# Autodesk Inventor assembly: Walls
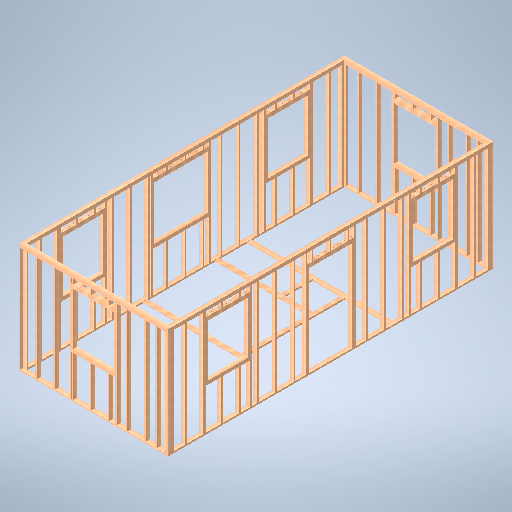
[picture p0: Inventor's stored thumbnail of the model, 512x512]
Saved by Autodesk Inventor 2025.1 (Build 291241020, 241B)
## iProperties
Created: 2024-09-15
Part Number: Walls
Document SubType Name: Assembly
Designer: Tom
Author: Tom
## Documents named in this file (17)
- C:\Users\Tom\Documents\Inventor\Mobility\Additional_Building\Framing_For_First_Floor.iam
- C:\Users\Tom\Documents\Inventor\Mobility\Additional_Building\Plate_With_Length_144_Inches.ipt
- C:\Users\Tom\Documents\Inventor\Mobility\Additional_Building\Plate_With_Length_125_Inches.ipt
- C:\Users\Tom\Documents\Inventor\Mobility\Additional_Building\California_Corner.iam
- C:\Users\Tom\Documents\Inventor\Mobility\Additional_Building\Stud_With_Height_93_Inches.ipt
- C:\Users\Tom\Documents\Inventor\Mobility\Additional_Building\Plate_With_Length_132_Inches.ipt
- C:\Users\Tom\Documents\Inventor\Mobility\Additional_Building\Plate_With_Length_68.5_Inches.ipt
- C:\Users\Tom\Documents\Inventor\Mobility\Additional_Building\Plate_With_Length_86.5625_Inches_And_Image_Of_Bath_Tub.ipt
- C:\Users\Tom\Documents\Inventor\Mobility\Additional_Building\Plate_With_Length_60_Inches.ipt
- C:\Users\Tom\Documents\Inventor\Mobility\Additional_Building\Plate_With_Length_25_Inches.ipt
- C:\Users\Tom\Documents\Inventor\Mobility\Additional_Building\Plate_With_Length_86.5625_Inches.ipt
- C:\Users\Tom\Documents\Inventor\Mobility\Additional_Building\Stud_With_Height_80.5_Inches.ipt
- C:\Users\Tom\Documents\Inventor\Mobility\Additional_Building\Stud_With_Height_9_Inches.ipt
- C:\Users\Tom\Documents\Inventor\Mobility\Additional_Building\Framing_For_First_Floor_Window.iam
- C:\Users\Tom\Documents\Inventor\Mobility\Additional_Building\Framing_For_Side_Window.iam
- C:\Users\Tom\Documents\Inventor\Mobility\Additional_Building\Framing_For_Bathroom_Window.iam
- C:\Users\Tom\Documents\Inventor\Mobility\Additional_Building\Header_With_Dimensions_3.5_x_3.5_x_41.25_Inches.iam
## Components (75 placed, 16 different names)
1. California_Corner:1 [sub-assembly] — Mate:2, Flush:3, Flush:4, Flush:95
2. California_Corner:2 [sub-assembly] — Mate:13, Flush:13, Flush:14, Flush:19, Flush:20, Flush:31, Mate:34, Flush:64, Flush:70
3. California_Corner:3 [sub-assembly] — Mate:14, Flush:15, Flush:16
4. California_Corner:4 [sub-assembly] — Mate:15, Flush:17, Flush:18
5. Plate_With_Length_125_Inches:5 — Mate:16, Flush:22, Mate:17, Mate:19, Mate:24, Flush:27, Flush:45
6. Plate_With_Length_60_Inches:1 — Mate:19, Mate:27, Mate:31, Flush:44
7. Plate_With_Length_25_Inches:1 — Mate:25, Mate:28, Flush:45
8. Plate_With_Length_25_Inches:2 — Mate:24, Flush:27, Mate:25, Mate:29
9. Plate_With_Length_86.5625_Inches_And_Image_Of_Bath_Tub:1 — Mate:26, Flush:28, Mate:27, Mate:28, Mate:29, Flush:44
10. Plate_With_Length_86.5625_Inches:1 — Mate:30, Mate:31, Flush:29, Mate:79
11. Stud_With_Height_93_Inches:56 — Mate:33, Flush:32, Mate:34, Mate:39
12. Stud_With_Height_93_Inches:57 — Mate:36, Flush:35, Mate:41, Mate:80, Flush:87
13. Stud_With_Height_80.5_Inches:1 — Mate:38, Flush:36, Mate:39
14. Stud_With_Height_80.5_Inches:2 — Mate:40, Flush:37, Mate:41, Mate:81
15. Framing_For_Bathroom_Window:1 [sub-assembly] — Mate:78, Flush:86, Mate:79
16. Header_With_Dimensions_3.5_x_3.5_x_41.25_Inches:1 [sub-assembly] — Mate:80, Mate:81, Flush:87
17. Plate_With_Length_132_Inches:1 — Mate:8, Flush:9, Flush:10, Mate:10
18. Plate_With_Length_132_Inches:2
19. Plate_With_Length_144_Inches:9 — Mate:11, Mate:12, Flush:12
20. Plate_With_Length_144_Inches:10
21. Stud_With_Height_9_Inches:1 — Flush:39
22. Stud_With_Height_9_Inches:2
23. Stud_With_Height_9_Inches:3
24. Stud_With_Height_93_Inches:49 — Mate:32, Flush:30, Flush:31
25. Framing_For_Side_Window:1 [sub-assembly] — Mate:65, Flush:69, Flush:70
26. Stud_With_Height_93_Inches:71
27. Framing_For_Side_Window:2 [sub-assembly]
28. Stud_With_Height_93_Inches:1 — Mate:4, Flush:6, Flush:19, Flush:39, Flush:43, Flush:88
29. Stud_With_Height_93_Inches:89 — Mate:84, Flush:93, Mate:85
30. Framing_For_First_Floor_Window:1 [sub-assembly] — Mate:62, Flush:63, Flush:64, Mate:85
31. Framing_For_First_Floor_Window:2 [sub-assembly] — Flush:94, Mate:86, Flush:95, Mate:88, Flush:98
32. Stud_With_Height_93_Inches:90 — Mate:87, Flush:96, Mate:88
33. Stud_With_Height_93_Inches:91 — Mate:89, Flush:97, Flush:98
34. Stud_With_Height_93_Inches:92
35. Stud_With_Height_93_Inches:93
36. Framing_For_First_Floor_Window:3 [sub-assembly]
37. Framing_For_First_Floor_Window:4 [sub-assembly]
38. Stud_With_Height_93_Inches:94
39. Stud_With_Height_93_Inches:95
40. Plate_With_Length_144_Inches:1 — Flush:5, Mate:15, Flush:17, Flush:18, Mate:30, Flush:29, Mate:78, Flush:86
41. Plate_With_Length_144_Inches:2 — Mate:14, Flush:15, Flush:16, Mate:26, Flush:28
42. Plate_With_Length_144_Inches:3 — Mate:1, Flush:1, Flush:2, Mate:4, Flush:6, Mate:13, Flush:13, Flush:14, Mate:16, Flush:22, Mate:33, Flush:32, Mate:38, Flush:36, Mate:61, Flush:61, Mate:62, Flush:63, Mate:84, Flush:93
43. Plate_With_Length_144_Inches:4 — Mate:2, Flush:3, Flush:4, Mate:36, Flush:35, Mate:40, Flush:37, Mate:44, Flush:42, Flush:94, Mate:86, Mate:87, Flush:96, Mate:89, Flush:97
44. Plate_With_Length_125_Inches:1 — Mate:1, Flush:1, Flush:2, Mate:3, Mate:7, Mate:32, Flush:30, Mate:65, Flush:69, Mate:66, Flush:71
45. Plate_With_Length_125_Inches:2 — Mate:17
46. Plate_With_Length_144_Inches:5 — Flush:9
47. Plate_With_Length_144_Inches:6
48. Plate_With_Length_144_Inches:7 — Mate:9, Flush:11
49. Plate_With_Length_144_Inches:8 — Mate:11, Flush:12
50. Plate_With_Length_125_Inches:3 — Flush:7, Mate:8, Flush:10
51. Plate_With_Length_125_Inches:4
52. Plate_With_Length_68.5_Inches:1 — Mate:9, Mate:10, Flush:11
53. Plate_With_Length_68.5_Inches:2 — Mate:12
54. Plate_With_Length_68.5_Inches:3
55. Plate_With_Length_68.5_Inches:4
56. Stud_With_Height_93_Inches:23 — Flush:7, Mate:7, Flush:20, Flush:72
57. Stud_With_Height_93_Inches:68
58. Stud_With_Height_93_Inches:69 — Mate:66, Flush:71, Flush:72
59. Stud_With_Height_93_Inches:70
60. Stud_With_Height_93_Inches:72
61. Stud_With_Height_93_Inches:73
62. Stud_With_Height_93_Inches:74
63. Stud_With_Height_93_Inches:75
64. Stud_With_Height_93_Inches:62 — Mate:61, Flush:61, Flush:88
65. Stud_With_Height_93_Inches:63
66. Stud_With_Height_93_Inches:85
67. Stud_With_Height_93_Inches:58 — Mate:44, Flush:42, Flush:43
68. Stud_With_Height_93_Inches:64
69. Stud_With_Height_93_Inches:86
70. Stud_With_Height_93_Inches:96
71. Stud_With_Height_93_Inches:97
72. Stud_With_Height_93_Inches:98
73. Stud_With_Height_93_Inches:99
74. Stud_With_Height_93_Inches:100
75. Stud_With_Height_93_Inches:101
## Component patterns: (2 elements), (2 elements, first: Plate_With_Length_132_Inches:1), (2 elements, first: Plate_With_Length_144_Inches:9), (3 elements, first: Stud_With_Height_9_Inches:1), (2 elements, first: Stud_With_Height_93_Inches:49 + Framing_For_Side_Window:1), (2 elements, first: Stud_With_Height_93_Inches:1 + Stud_With_Height_93_Inches:89 + Framing_For_First_Floor_Window:1 + Framing_For_First_Floor_Window:2 + Stud_With_Height_93_Inches:90 + Stud_With_Height_93_Inches:91), (4 elements, first: Plate_With_Length_144_Inches:1), (2 elements, first: Plate_With_Length_125_Inches:1), Component Pattern 1:2 (4 elements), Component Pattern 2:2 (2 elements), (2 elements, first: Plate_With_Length_68.5_Inches:1), Component Pattern 10:2 (2 elements), (2 elements, first: Stud_With_Height_93_Inches:23), (2 elements, first: Stud_With_Height_93_Inches:69), Component Pattern 22:2 (2 elements), Component Pattern 23:2 (2 elements), (3 elements, first: Stud_With_Height_93_Inches:62), (3 elements, first: Stud_With_Height_93_Inches:58), Component Pattern 19:2 (3 elements), Component Pattern 20:2 (3 elements)
## Relationships (97: Flush 50, Mate 47)
- Mate:1: Plate_With_Length_144_Inches:3 ↔ Plate_With_Length_125_Inches:1
- Flush:1: Plate_With_Length_144_Inches:3 ↔ Plate_With_Length_125_Inches:1
- Flush:2: Plate_With_Length_144_Inches:3 ↔ Plate_With_Length_125_Inches:1
- Mate:2: California_Corner:1 ↔ Plate_With_Length_144_Inches:4
- Flush:3: California_Corner:1 ↔ Plate_With_Length_144_Inches:4
- Flush:4: California_Corner:1 ↔ Plate_With_Length_144_Inches:4
- Flush:5: Plate_With_Length_144_Inches:1
- Mate:3 (1536.7 mm): Plate_With_Length_125_Inches:1
- Mate:4: Stud_With_Height_93_Inches:1 ↔ Plate_With_Length_144_Inches:3
- Flush:6: Stud_With_Height_93_Inches:1 ↔ Plate_With_Length_144_Inches:3
- Flush:7: Plate_With_Length_125_Inches:3 ↔ Stud_With_Height_93_Inches:23
- Mate:7: Plate_With_Length_125_Inches:1 ↔ Stud_With_Height_93_Inches:23
- Mate:8: Plate_With_Length_132_Inches:1 ↔ Plate_With_Length_125_Inches:3
- Flush:9: Plate_With_Length_132_Inches:1 ↔ Plate_With_Length_144_Inches:5
- Flush:10: Plate_With_Length_132_Inches:1 ↔ Plate_With_Length_125_Inches:3
- Mate:9: Plate_With_Length_144_Inches:7 ↔ Plate_With_Length_68.5_Inches:1
- Mate:10: Plate_With_Length_132_Inches:1 ↔ Plate_With_Length_68.5_Inches:1
- Flush:11: Plate_With_Length_144_Inches:7 ↔ Plate_With_Length_68.5_Inches:1
- Mate:11: Plate_With_Length_144_Inches:9 ↔ Plate_With_Length_144_Inches:8
- Mate:12: Plate_With_Length_144_Inches:9 ↔ Plate_With_Length_68.5_Inches:2
- Flush:12: Plate_With_Length_144_Inches:9 ↔ Plate_With_Length_144_Inches:8
- Mate:13: California_Corner:2 ↔ Plate_With_Length_144_Inches:3
- Flush:13: California_Corner:2 ↔ Plate_With_Length_144_Inches:3
- Flush:14: California_Corner:2 ↔ Plate_With_Length_144_Inches:3
- Mate:14: California_Corner:3 ↔ Plate_With_Length_144_Inches:2
- Flush:15: California_Corner:3 ↔ Plate_With_Length_144_Inches:2
- Flush:16: California_Corner:3 ↔ Plate_With_Length_144_Inches:2
- Mate:15: California_Corner:4 ↔ Plate_With_Length_144_Inches:1
- Flush:17: California_Corner:4 ↔ Plate_With_Length_144_Inches:1
- Flush:18: California_Corner:4 ↔ Plate_With_Length_144_Inches:1
- Flush:19 (387.35 mm): California_Corner:2 ↔ Stud_With_Height_93_Inches:1
- Flush:20 (501.65 mm): California_Corner:2 ↔ Stud_With_Height_93_Inches:23
- Mate:16: Plate_With_Length_125_Inches:5 ↔ Plate_With_Length_144_Inches:3
- Flush:22: Plate_With_Length_125_Inches:5 ↔ Plate_With_Length_144_Inches:3
- Mate:17 (2092.325 mm): Plate_With_Length_125_Inches:5 ↔ Plate_With_Length_125_Inches:2
- Mate:19 (723.9 mm): Plate_With_Length_125_Inches:5 ↔ Plate_With_Length_60_Inches:1
- Mate:24: Plate_With_Length_125_Inches:5 ↔ Plate_With_Length_25_Inches:2
- Flush:27: Plate_With_Length_125_Inches:5 ↔ Plate_With_Length_25_Inches:2
- Mate:25 (635 mm): Plate_With_Length_25_Inches:1 ↔ Plate_With_Length_25_Inches:2
- Mate:26: Plate_With_Length_86.5625_Inches_And_Image_Of_Bath_Tub:1 ↔ Plate_With_Length_144_Inches:2
- Flush:28: Plate_With_Length_86.5625_Inches_And_Image_Of_Bath_Tub:1 ↔ Plate_With_Length_144_Inches:2
- Mate:27: Plate_With_Length_60_Inches:1 ↔ Plate_With_Length_86.5625_Inches_And_Image_Of_Bath_Tub:1
- Mate:28: Plate_With_Length_25_Inches:1 ↔ Plate_With_Length_86.5625_Inches_And_Image_Of_Bath_Tub:1
- Mate:29: Plate_With_Length_25_Inches:2 ↔ Plate_With_Length_86.5625_Inches_And_Image_Of_Bath_Tub:1
- Mate:30: Plate_With_Length_86.5625_Inches:1 ↔ Plate_With_Length_144_Inches:1
- Mate:31: Plate_With_Length_60_Inches:1 ↔ Plate_With_Length_86.5625_Inches:1
- Flush:29: Plate_With_Length_86.5625_Inches:1 ↔ Plate_With_Length_144_Inches:1
- Mate:32: Stud_With_Height_93_Inches:49 ↔ Plate_With_Length_125_Inches:1
- Flush:30: Stud_With_Height_93_Inches:49 ↔ Plate_With_Length_125_Inches:1
- Flush:31 (250.825 mm): California_Corner:2 ↔ Stud_With_Height_93_Inches:49
- Mate:33: Stud_With_Height_93_Inches:56 ↔ Plate_With_Length_144_Inches:3
- Flush:32: Stud_With_Height_93_Inches:56 ↔ Plate_With_Length_144_Inches:3
- Mate:34 (-3133.725 mm): California_Corner:2 ↔ Stud_With_Height_93_Inches:56
- Mate:36: Stud_With_Height_93_Inches:57 ↔ Plate_With_Length_144_Inches:4
- Flush:35: Stud_With_Height_93_Inches:57 ↔ Plate_With_Length_144_Inches:4
- Mate:38: Stud_With_Height_80.5_Inches:1 ↔ Plate_With_Length_144_Inches:3
- Flush:36: Stud_With_Height_80.5_Inches:1 ↔ Plate_With_Length_144_Inches:3
- Mate:39: Stud_With_Height_93_Inches:56 ↔ Stud_With_Height_80.5_Inches:1
- Mate:40: Stud_With_Height_80.5_Inches:2 ↔ Plate_With_Length_144_Inches:4
- Flush:37: Stud_With_Height_80.5_Inches:2 ↔ Plate_With_Length_144_Inches:4
- Mate:41: Stud_With_Height_93_Inches:57 ↔ Stud_With_Height_80.5_Inches:2
- Flush:39 (2844.8 mm): Stud_With_Height_9_Inches:1 ↔ Stud_With_Height_93_Inches:1
- Mate:44: Plate_With_Length_144_Inches:4 ↔ Stud_With_Height_93_Inches:58
- Flush:42: Plate_With_Length_144_Inches:4 ↔ Stud_With_Height_93_Inches:58
- Flush:43 (4064 mm): Stud_With_Height_93_Inches:1 ↔ Stud_With_Height_93_Inches:58
- Flush:44: Plate_With_Length_60_Inches:1 ↔ Plate_With_Length_86.5625_Inches_And_Image_Of_Bath_Tub:1
- Flush:45: Plate_With_Length_125_Inches:5 ↔ Plate_With_Length_25_Inches:1
- Mate:61: Plate_With_Length_144_Inches:3 ↔ Stud_With_Height_93_Inches:62
- Flush:61: Plate_With_Length_144_Inches:3 ↔ Stud_With_Height_93_Inches:62
- Mate:62: Framing_For_First_Floor_Window:1 ↔ Plate_With_Length_144_Inches:3
- Flush:63: Framing_For_First_Floor_Window:1 ↔ Plate_With_Length_144_Inches:3
- Flush:64 (820.7375 mm): California_Corner:2 ↔ Framing_For_First_Floor_Window:1
- Mate:65: Framing_For_Side_Window:1 ↔ Plate_With_Length_125_Inches:1
- Flush:69: Framing_For_Side_Window:1 ↔ Plate_With_Length_125_Inches:1
- Flush:70 (1143 mm): California_Corner:2 ↔ Framing_For_Side_Window:1
- Mate:66: Plate_With_Length_125_Inches:1 ↔ Stud_With_Height_93_Inches:69
- Flush:71: Plate_With_Length_125_Inches:1 ↔ Stud_With_Height_93_Inches:69
- Flush:72 (2032 mm): Stud_With_Height_93_Inches:23 ↔ Stud_With_Height_93_Inches:69
- Mate:78: Framing_For_Bathroom_Window:1 ↔ Plate_With_Length_144_Inches:1
- Flush:86: Framing_For_Bathroom_Window:1 ↔ Plate_With_Length_144_Inches:1
- Mate:79 (85.725 mm): Plate_With_Length_86.5625_Inches:1 ↔ Framing_For_Bathroom_Window:1
- Mate:80: Stud_With_Height_93_Inches:57 ↔ Header_With_Dimensions_3.5_x_3.5_x_41.25_Inches:1
- Mate:81: Stud_With_Height_80.5_Inches:2 ↔ Header_With_Dimensions_3.5_x_3.5_x_41.25_Inches:1
- Flush:87: Stud_With_Height_93_Inches:57 ↔ Header_With_Dimensions_3.5_x_3.5_x_41.25_Inches:1
- Flush:88 (1625.6 mm): Stud_With_Height_93_Inches:1 ↔ Stud_With_Height_93_Inches:62
- Mate:84: Stud_With_Height_93_Inches:89 ↔ Plate_With_Length_144_Inches:3
- Flush:93: Stud_With_Height_93_Inches:89 ↔ Plate_With_Length_144_Inches:3
- Mate:85: Stud_With_Height_93_Inches:89 ↔ Framing_For_First_Floor_Window:1
- Flush:94: Framing_For_First_Floor_Window:2 ↔ Plate_With_Length_144_Inches:4
- Mate:86: Framing_For_First_Floor_Window:2 ↔ Plate_With_Length_144_Inches:4
- Flush:95 (820.7375 mm): California_Corner:1 ↔ Framing_For_First_Floor_Window:2
- Mate:87: Stud_With_Height_93_Inches:90 ↔ Plate_With_Length_144_Inches:4
- Flush:96: Stud_With_Height_93_Inches:90 ↔ Plate_With_Length_144_Inches:4
- Mate:88: Framing_For_First_Floor_Window:2 ↔ Stud_With_Height_93_Inches:90
- Mate:89: Stud_With_Height_93_Inches:91 ↔ Plate_With_Length_144_Inches:4
- Flush:97: Stud_With_Height_93_Inches:91 ↔ Plate_With_Length_144_Inches:4
- Flush:98 (812.8 mm): Framing_For_First_Floor_Window:2 ↔ Stud_With_Height_93_Inches:91
